# Autodesk Inventor assembly: Shooter Curve Assembly
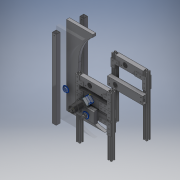
[picture p0: Inventor's stored thumbnail of the model, 180x180]
Saved by Autodesk Inventor 2018 (Build 220112000, 112)
## iProperties
Created: 2020-02-01
Part Number: Shooter Curve Assembly
Document SubType Name: Assembly
Designer: Weeb No1
Author: Weeb No1
## Documents named in this file (14)
- C:\Users\T3500STATIC\Documents\GitHub\2020CAD\Gabriel Inventor Files (Shooter, Drivebase)\Shooter Curve Assembly\Main Assembly File\Shooter Curve Assembly.iam
- C:\Users\T3500STATIC\Documents\GitHub\2020CAD\Gabriel Inventor Files (Shooter, Drivebase)\Shooter Curve Assembly\Part Files\Shooter Main Curve.ipt
- C:\Users\T3500STATIC\Documents\GitHub\2020CAD\Gabriel Inventor Files (Shooter, Drivebase)\Shooter Curve Assembly\Part Files\8020 1010 x 15.ipt
- C:\Users\T3500STATIC\Documents\GitHub\2020CAD\Gabriel Inventor Files (Shooter, Drivebase)\Shooter Curve Assembly\Part Files\1x2 5 in Beam Flywheel Mount.ipt
- C:\Users\T3500STATIC\Documents\GitHub\2020CAD\Over bumper intake\Parts\VersaPlanetary_v2_Single_Stage_10_1_with_775_Series.iam
- C:\Users\T3500STATIC\Documents\GitHub\2020CAD\Gabriel Inventor Files (Shooter, Drivebase)\Shooter Curve Assembly\Part Files\1x2 7 in Beam Motor Mount.ipt
- C:\Users\T3500STATIC\Documents\GitHub\2020CAD\Gabriel Inventor Files (Shooter, Drivebase)\Gussets\L-Gusset 3 Hole 0.25in Hole.ipt
- C:\Users\T3500STATIC\Documents\GitHub\2020CAD\Gabriel Inventor Files (Shooter, Drivebase)\Shooter Curve Assembly\Part Files\1x1 20 in Curve Support Beam.ipt
- C:\Users\T3500STATIC\Documents\GitHub\2020CAD\Gabriel Inventor Files (Shooter, Drivebase)\Gussets\L-Guesset 4 Hole 0.25in Hole.ipt
- C:\Users\T3500STATIC\Documents\GitHub\2020CAD\Gabriel Inventor Files (Shooter, Drivebase)\Gussets\L-Guesset 5 Hole 0.25in Hole.ipt
- C:\Users\T3500STATIC\Documents\GitHub\2020CAD\Gabriel Inventor Files (Shooter, Drivebase)\Shooter Curve Assembly\Part Files\_18t_Aluminum_Hub_Sprocket_25_Chain_1_2_Hex_Bore_217-3488.ipt
- C:\Users\T3500STATIC\Documents\GitHub\2020CAD\Gabriel Inventor Files (Shooter, Drivebase)\Shooter Curve Assembly\Part Files\Top Conveyor Roller Wheel Assembly.iam
- C:\Users\T3500STATIC\Documents\GitHub\2020CAD\Gabriel Inventor Files (Shooter, Drivebase)\Gussets\2in 4-hole Bracket 0.25in Hole.ipt
- C:\Users\T3500STATIC\Documents\GitHub\2020CAD\Gabriel Inventor Files (Shooter, Drivebase)\Shooter Curve Assembly\Part Files\Roller Wheel Right Side Support Beam.ipt
## Components (34 placed, 13 different names)
1. Shooter Main Curve:1 — Flush:1, Mate:1, Mate:2, Flush:2, Flush:3, Flush:18, Flush:20, Mate:68, Flush:36, Flush:37, Flush:40, Flush:41, Mate:133
2. 8020 1010 x 15:1 — Flush:1, Mate:1, Flush:5, Flush:6, Mate:7, Flush:11, Flush:14, Flush:18, Flush:23, Flush:24, Mate:51, Mate:56, Mate:60, Mate:82, Mate:85, Mate:97, Mate:100, Flush:44, Flush:45, Mate:145, Flush:47, Flush:49, Mate:151, Flush:50
3. 8020 1010 x 15:2 — Flush:4, Mate:3, Flush:7, Mate:9, Flush:15, Flush:19, Flush:22, Flush:25, Mate:127, Mate:130, Mate:156, Flush:52
4. Shooter Main Curve:2 — Mate:2, Flush:2, Flush:3, Flush:4, Mate:3, Flush:19, Flush:21, Mate:67, Flush:35, Flush:38, Flush:39, Mate:132
5. 8020 1010 x 15:3 — Flush:5, Flush:6, Flush:10, Flush:12, Flush:13, Flush:20, Mate:11, Flush:23, Mate:50, Flush:34, Mate:63, Mate:65, Mate:89, Mate:93, Mate:103, Mate:123, Flush:42, Flush:43, Mate:140, Mate:144, Flush:46, Flush:48
6. 8020 1010 x 15:4 — Flush:7, Flush:10, Flush:17, Flush:21, Mate:10, Flush:22, Mate:107, Mate:111, Mate:155, Flush:51
7. 1x2 5 in Beam Flywheel Mount:1 — Mate:9, Flush:15, Flush:17, Mate:10, Flush:25, Mate:106, Mate:108, Mate:109, Mate:110, Mate:112, Mate:113, Mate:126, Mate:128, Mate:129, Mate:131
8. 1x2 5 in Beam Flywheel Mount:2 — Mate:7, Flush:11, Flush:12, Flush:13, Flush:14, Mate:11, Flush:24, Mate:55, Mate:58, Mate:61, Mate:64, Mate:134, Mate:135, Mate:136, Mate:137
9. VersaPlanetary_v2_Single_Stage_10_1_with_775_Series:1 [sub-assembly] — Mate:52, Mate:53, Mate:54
10. 1x2 7 in Beam Motor Mount:1 — Mate:50, Mate:51, Flush:34, Mate:52, Mate:53, Mate:54, Mate:81, Mate:86, Mate:88, Mate:90, Mate:91, Mate:92, Mate:94, Mate:95, Mate:96, Mate:98, Mate:99, Mate:101, Mate:102, Mate:122, Mate:141, Mate:142, Mate:143, Mate:146, Mate:149, Mate:150
11. L-Gusset 3 Hole 0.25in Hole:1 — Mate:61, Mate:63, Mate:137, Flush:42
12. L-Gusset 3 Hole 0.25in Hole:2 — Mate:55, Mate:56, Mate:135, Flush:44, Mate:139
13. L-Gusset 3 Hole 0.25in Hole:3 — Mate:58, Mate:60, Mate:134, Flush:45
14. L-Gusset 3 Hole 0.25in Hole:4 — Mate:64, Mate:65, Mate:136, Flush:43, Mate:138
15. 1x1 20 in Curve Support Beam:1 — Mate:68, Flush:36, Flush:37
16. 1x1 20 in Curve Support Beam:2 — Mate:67, Flush:35, Flush:38
17. L-Guesset 4 Hole 0.25in Hole:3 — Mate:88, Mate:89, Mate:90, Mate:91
18. L-Guesset 4 Hole 0.25in Hole:5 — Mate:81, Mate:82, Mate:150
19. L-Guesset 4 Hole 0.25in Hole:6 — Mate:85, Mate:86, Mate:149
20. L-Guesset 4 Hole 0.25in Hole:9 — Mate:92, Mate:93, Mate:94, Mate:95, Mate:138
21. L-Gusset 3 Hole 0.25in Hole:9 — Mate:96, Mate:97, Mate:98, Mate:139
22. L-Gusset 3 Hole 0.25in Hole:10 — Mate:99, Mate:100, Mate:101
23. L-Guesset 5 Hole 0.25in Hole:1 — Mate:102, Mate:103
24. L-Guesset 5 Hole 0.25in Hole:2 — Mate:110, Mate:111, Mate:112, Mate:113
25. L-Guesset 5 Hole 0.25in Hole:3 — Mate:106, Mate:107, Mate:108, Mate:109
26. L-Guesset 5 Hole 0.25in Hole:6 — Mate:122, Mate:123, Mate:147, Mate:148
27. L-Gusset 3 Hole 0.25in Hole:11 — Mate:126, Mate:127, Mate:128
28. L-Gusset 3 Hole 0.25in Hole:12 — Mate:129, Mate:130, Mate:131
29. _18t_Aluminum_Hub_Sprocket_25_Chain_1_2_Hex_Bore_217-3488:1
30. Shooter Main Curve:4 — Flush:39, Flush:40, Flush:41, Mate:132, Mate:133
31. L-Guesset 4 Hole 0.25in Hole:10 — Mate:140, Mate:141, Mate:142, Mate:143
32. Top Conveyor Roller Wheel Assembly:1 [sub-assembly] — Mate:144, Mate:145, Flush:46, Flush:47, Flush:48, Flush:49, Mate:146, Mate:147, Mate:148, Mate:152, Mate:153, Mate:154
33. 2in 4-hole Bracket 0.25in Hole:1 — Mate:151, Mate:152, Mate:153, Mate:154, Flush:50
34. Roller Wheel Right Side Support Beam:1 — Mate:155, Mate:156, Flush:51, Flush:52
## Relationships (124: Mate 83, Flush 41)
- Flush:1 (177.8 mm): Shooter Main Curve:1 ↔ 8020 1010 x 15:1
- Mate:1 (25.4 mm): Shooter Main Curve:1 ↔ 8020 1010 x 15:1
- Mate:2 (114.3 mm): Shooter Main Curve:1 ↔ Shooter Main Curve:2
- Flush:2: Shooter Main Curve:1 ↔ Shooter Main Curve:2
- Flush:3: Shooter Main Curve:1 ↔ Shooter Main Curve:2
- Flush:4 (177.8 mm): 8020 1010 x 15:2 ↔ Shooter Main Curve:2
- Mate:3 (25.4 mm): 8020 1010 x 15:2 ↔ Shooter Main Curve:2
- Flush:5: 8020 1010 x 15:1 ↔ 8020 1010 x 15:3
- Flush:6: 8020 1010 x 15:1 ↔ 8020 1010 x 15:3
- Flush:7: 8020 1010 x 15:2 ↔ 8020 1010 x 15:4
- Flush:10: 8020 1010 x 15:3 ↔ 8020 1010 x 15:4
- Mate:7: 8020 1010 x 15:1 ↔ 1x2 5 in Beam Flywheel Mount:2
- Flush:11: 8020 1010 x 15:1 ↔ 1x2 5 in Beam Flywheel Mount:2
- Flush:12: 8020 1010 x 15:3 ↔ 1x2 5 in Beam Flywheel Mount:2
- Flush:13: 8020 1010 x 15:3 ↔ 1x2 5 in Beam Flywheel Mount:2
- Flush:14: 8020 1010 x 15:1 ↔ 1x2 5 in Beam Flywheel Mount:2
- Mate:9: 8020 1010 x 15:2 ↔ 1x2 5 in Beam Flywheel Mount:1
- Flush:15: 8020 1010 x 15:2 ↔ 1x2 5 in Beam Flywheel Mount:1
- Flush:17: 8020 1010 x 15:4 ↔ 1x2 5 in Beam Flywheel Mount:1
- Flush:18 (-25.4 mm): Shooter Main Curve:1 ↔ 8020 1010 x 15:1
- Flush:19 (-25.4 mm): 8020 1010 x 15:2 ↔ Shooter Main Curve:2
- Flush:20 (-25.4 mm): Shooter Main Curve:1 ↔ 8020 1010 x 15:3
- Flush:21 (-25.4 mm): Shooter Main Curve:2 ↔ 8020 1010 x 15:4
- Mate:10: 8020 1010 x 15:4 ↔ 1x2 5 in Beam Flywheel Mount:1
- Mate:11: 8020 1010 x 15:3 ↔ 1x2 5 in Beam Flywheel Mount:2
- Flush:22: 8020 1010 x 15:2 ↔ 8020 1010 x 15:4
- Flush:23: 8020 1010 x 15:1 ↔ 8020 1010 x 15:3
- Flush:24: 8020 1010 x 15:1 ↔ 1x2 5 in Beam Flywheel Mount:2
- Flush:25: 8020 1010 x 15:2 ↔ 1x2 5 in Beam Flywheel Mount:1
- Mate:50: 8020 1010 x 15:3 ↔ 1x2 7 in Beam Motor Mount:1
- Mate:51: 8020 1010 x 15:1 ↔ 1x2 7 in Beam Motor Mount:1
- Flush:34: 8020 1010 x 15:3 ↔ 1x2 7 in Beam Motor Mount:1
- Mate:52: VersaPlanetary_v2_Single_Stage_10_1_with_775_Series:1 ↔ 1x2 7 in Beam Motor Mount:1
- Mate:53: VersaPlanetary_v2_Single_Stage_10_1_with_775_Series:1 ↔ 1x2 7 in Beam Motor Mount:1
- Mate:54: VersaPlanetary_v2_Single_Stage_10_1_with_775_Series:1 ↔ 1x2 7 in Beam Motor Mount:1
- Mate:55: 1x2 5 in Beam Flywheel Mount:2 ↔ L-Gusset 3 Hole 0.25in Hole:2
- Mate:56: 8020 1010 x 15:1 ↔ L-Gusset 3 Hole 0.25in Hole:2
- Mate:58: 1x2 5 in Beam Flywheel Mount:2 ↔ L-Gusset 3 Hole 0.25in Hole:3
- Mate:60: 8020 1010 x 15:1 ↔ L-Gusset 3 Hole 0.25in Hole:3
- Mate:61: 1x2 5 in Beam Flywheel Mount:2 ↔ L-Gusset 3 Hole 0.25in Hole:1
- Mate:63: 8020 1010 x 15:3 ↔ L-Gusset 3 Hole 0.25in Hole:1
- Mate:64: 1x2 5 in Beam Flywheel Mount:2 ↔ L-Gusset 3 Hole 0.25in Hole:4
- Mate:65: 8020 1010 x 15:3 ↔ L-Gusset 3 Hole 0.25in Hole:4
- Mate:67: Shooter Main Curve:2 ↔ 1x1 20 in Curve Support Beam:2
- Flush:35 (-25.4 mm): Shooter Main Curve:2 ↔ 1x1 20 in Curve Support Beam:2
- Mate:68: Shooter Main Curve:1 ↔ 1x1 20 in Curve Support Beam:1
- Flush:36 (-25.4 mm): Shooter Main Curve:1 ↔ 1x1 20 in Curve Support Beam:1
- Flush:37: Shooter Main Curve:1 ↔ 1x1 20 in Curve Support Beam:1
- Flush:38: Shooter Main Curve:2 ↔ 1x1 20 in Curve Support Beam:2
- Mate:81: 1x2 7 in Beam Motor Mount:1 ↔ L-Guesset 4 Hole 0.25in Hole:5
- Mate:82: 8020 1010 x 15:1 ↔ L-Guesset 4 Hole 0.25in Hole:5
- Mate:85: 8020 1010 x 15:1 ↔ L-Guesset 4 Hole 0.25in Hole:6
- Mate:86: 1x2 7 in Beam Motor Mount:1 ↔ L-Guesset 4 Hole 0.25in Hole:6
- Mate:88: 1x2 7 in Beam Motor Mount:1 ↔ L-Guesset 4 Hole 0.25in Hole:3
- Mate:89: 8020 1010 x 15:3 ↔ L-Guesset 4 Hole 0.25in Hole:3
- Mate:90: 1x2 7 in Beam Motor Mount:1 ↔ L-Guesset 4 Hole 0.25in Hole:3
- Mate:91: 1x2 7 in Beam Motor Mount:1 ↔ L-Guesset 4 Hole 0.25in Hole:3
- Mate:92: 1x2 7 in Beam Motor Mount:1 ↔ L-Guesset 4 Hole 0.25in Hole:9
- Mate:93: 8020 1010 x 15:3 ↔ L-Guesset 4 Hole 0.25in Hole:9
- Mate:94: 1x2 7 in Beam Motor Mount:1 ↔ L-Guesset 4 Hole 0.25in Hole:9
- Mate:95: 1x2 7 in Beam Motor Mount:1 ↔ L-Guesset 4 Hole 0.25in Hole:9
- Mate:96: 1x2 7 in Beam Motor Mount:1 ↔ L-Gusset 3 Hole 0.25in Hole:9
- Mate:97: 8020 1010 x 15:1 ↔ L-Gusset 3 Hole 0.25in Hole:9
- Mate:98: 1x2 7 in Beam Motor Mount:1 ↔ L-Gusset 3 Hole 0.25in Hole:9
- Mate:99: 1x2 7 in Beam Motor Mount:1 ↔ L-Gusset 3 Hole 0.25in Hole:10
- Mate:100: 8020 1010 x 15:1 ↔ L-Gusset 3 Hole 0.25in Hole:10
- Mate:101: 1x2 7 in Beam Motor Mount:1 ↔ L-Gusset 3 Hole 0.25in Hole:10
- Mate:102: 1x2 7 in Beam Motor Mount:1 ↔ L-Guesset 5 Hole 0.25in Hole:1
- Mate:103: 8020 1010 x 15:3 ↔ L-Guesset 5 Hole 0.25in Hole:1
- Mate:106: 1x2 5 in Beam Flywheel Mount:1 ↔ L-Guesset 5 Hole 0.25in Hole:3
- Mate:107: 8020 1010 x 15:4 ↔ L-Guesset 5 Hole 0.25in Hole:3
- Mate:108: 1x2 5 in Beam Flywheel Mount:1 ↔ L-Guesset 5 Hole 0.25in Hole:3
- Mate:109: 1x2 5 in Beam Flywheel Mount:1 ↔ L-Guesset 5 Hole 0.25in Hole:3
- Mate:110: 1x2 5 in Beam Flywheel Mount:1 ↔ L-Guesset 5 Hole 0.25in Hole:2
- Mate:111: 8020 1010 x 15:4 ↔ L-Guesset 5 Hole 0.25in Hole:2
- Mate:112: 1x2 5 in Beam Flywheel Mount:1 ↔ L-Guesset 5 Hole 0.25in Hole:2
- Mate:113: 1x2 5 in Beam Flywheel Mount:1 ↔ L-Guesset 5 Hole 0.25in Hole:2
- Mate:122: 1x2 7 in Beam Motor Mount:1 ↔ L-Guesset 5 Hole 0.25in Hole:6
- Mate:123: 8020 1010 x 15:3 ↔ L-Guesset 5 Hole 0.25in Hole:6
- Mate:126: 1x2 5 in Beam Flywheel Mount:1 ↔ L-Gusset 3 Hole 0.25in Hole:11
- Mate:127: 8020 1010 x 15:2 ↔ L-Gusset 3 Hole 0.25in Hole:11
- Mate:128: 1x2 5 in Beam Flywheel Mount:1 ↔ L-Gusset 3 Hole 0.25in Hole:11
- Mate:129: 1x2 5 in Beam Flywheel Mount:1 ↔ L-Gusset 3 Hole 0.25in Hole:12
- Mate:130: 8020 1010 x 15:2 ↔ L-Gusset 3 Hole 0.25in Hole:12
- Mate:131: 1x2 5 in Beam Flywheel Mount:1 ↔ L-Gusset 3 Hole 0.25in Hole:12
- Flush:39: Shooter Main Curve:2 ↔ Shooter Main Curve:4
- Flush:40: Shooter Main Curve:1 ↔ Shooter Main Curve:4
- Flush:41: Shooter Main Curve:1 ↔ Shooter Main Curve:4
- Mate:132 (47.625 mm): Shooter Main Curve:2 ↔ Shooter Main Curve:4
- Mate:133 (47.625 mm): Shooter Main Curve:1 ↔ Shooter Main Curve:4
- Mate:134: 1x2 5 in Beam Flywheel Mount:2 ↔ L-Gusset 3 Hole 0.25in Hole:3
- Mate:135: 1x2 5 in Beam Flywheel Mount:2 ↔ L-Gusset 3 Hole 0.25in Hole:2
- Mate:136: 1x2 5 in Beam Flywheel Mount:2 ↔ L-Gusset 3 Hole 0.25in Hole:4
- Mate:137: 1x2 5 in Beam Flywheel Mount:2 ↔ L-Gusset 3 Hole 0.25in Hole:1
- Flush:42: 8020 1010 x 15:3 ↔ L-Gusset 3 Hole 0.25in Hole:1
- Flush:43: 8020 1010 x 15:3 ↔ L-Gusset 3 Hole 0.25in Hole:4
- Flush:44: 8020 1010 x 15:1 ↔ L-Gusset 3 Hole 0.25in Hole:2
- Flush:45: 8020 1010 x 15:1 ↔ L-Gusset 3 Hole 0.25in Hole:3
- Mate:138: L-Gusset 3 Hole 0.25in Hole:4 ↔ L-Guesset 4 Hole 0.25in Hole:9
- Mate:139: L-Gusset 3 Hole 0.25in Hole:2 ↔ L-Gusset 3 Hole 0.25in Hole:9
- Mate:140: 8020 1010 x 15:3 ↔ L-Guesset 4 Hole 0.25in Hole:10
- Mate:141: 1x2 7 in Beam Motor Mount:1 ↔ L-Guesset 4 Hole 0.25in Hole:10
- Mate:142: 1x2 7 in Beam Motor Mount:1 ↔ L-Guesset 4 Hole 0.25in Hole:10
- Mate:143: 1x2 7 in Beam Motor Mount:1 ↔ L-Guesset 4 Hole 0.25in Hole:10
- Mate:144: 8020 1010 x 15:3 ↔ Top Conveyor Roller Wheel Assembly:1
- Mate:145: 8020 1010 x 15:1 ↔ Top Conveyor Roller Wheel Assembly:1
- Flush:46: 8020 1010 x 15:3 ↔ Top Conveyor Roller Wheel Assembly:1
- Flush:47: 8020 1010 x 15:1 ↔ Top Conveyor Roller Wheel Assembly:1
- Flush:48: 8020 1010 x 15:3 ↔ Top Conveyor Roller Wheel Assembly:1
- Flush:49: 8020 1010 x 15:1 ↔ Top Conveyor Roller Wheel Assembly:1
- Mate:146 (12.7 mm): 1x2 7 in Beam Motor Mount:1 ↔ Top Conveyor Roller Wheel Assembly:1
- Mate:147: L-Guesset 5 Hole 0.25in Hole:6 ↔ Top Conveyor Roller Wheel Assembly:1
- Mate:148: L-Guesset 5 Hole 0.25in Hole:6 ↔ Top Conveyor Roller Wheel Assembly:1
- Mate:149: 1x2 7 in Beam Motor Mount:1 ↔ L-Guesset 4 Hole 0.25in Hole:6
- Mate:150: 1x2 7 in Beam Motor Mount:1 ↔ L-Guesset 4 Hole 0.25in Hole:5
- Mate:151: 8020 1010 x 15:1 ↔ 2in 4-hole Bracket 0.25in Hole:1
- Mate:152: Top Conveyor Roller Wheel Assembly:1 ↔ 2in 4-hole Bracket 0.25in Hole:1
- Mate:153: Top Conveyor Roller Wheel Assembly:1 ↔ 2in 4-hole Bracket 0.25in Hole:1
- Mate:154: Top Conveyor Roller Wheel Assembly:1 ↔ 2in 4-hole Bracket 0.25in Hole:1
- Flush:50: 8020 1010 x 15:1 ↔ 2in 4-hole Bracket 0.25in Hole:1
- Mate:155: 8020 1010 x 15:4 ↔ Roller Wheel Right Side Support Beam:1
- Mate:156: 8020 1010 x 15:2 ↔ Roller Wheel Right Side Support Beam:1
- Flush:51: 8020 1010 x 15:4 ↔ Roller Wheel Right Side Support Beam:1
- Flush:52: 8020 1010 x 15:2 ↔ Roller Wheel Right Side Support Beam:1
